# Autodesk Inventor assembly: ヘラ
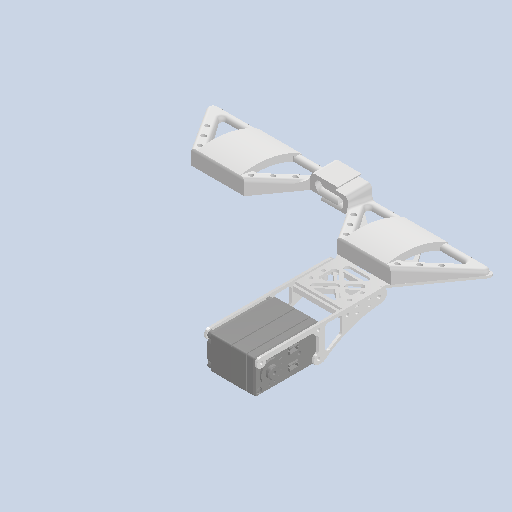
[picture p0: Inventor's stored thumbnail of the model, 512x512]
Saved by Autodesk Inventor 2024 (Build 280153000, 153)
## iProperties
Created: 2023-08-01
Part Number: ヘラ
Document SubType Name: Assembly
Designer: right
Mass: 56.6526 g
Surface Area: 176.367 cm^2
Volume: 31.3921 cm^3
Density: 1.80467 g/cm^3
Author: right
## Documents named in this file (7)
- C:\Users\right\OneDrive\ドキュメント\Inventor\V2二足Light＿仮\ヘラ.iam
- C:\Users\right\OneDrive\ドキュメント\Inventor\V2二足Light＿仮\KRS2500_scale.ipt
- C:\Users\right\OneDrive\ドキュメント\Inventor\V2二足Light＿仮\hera_nemoto.ipt
- C:\Users\right\OneDrive\ドキュメント\Inventor\V2二足Light＿仮\heraosae.ipt
- C:\Users\right\OneDrive\ドキュメント\Inventor\V2二足Light＿仮\hera.ipt
- C:\Users\right\OneDrive\ドキュメント\Inventor\V2二足Light＿仮\heraue_2.ipt
- C:\Users\right\OneDrive\ドキュメント\Inventor\V2二足Light＿仮\heraue_2_MIR.ipt
## Components (7 placed, 6 different names)
1. KRS2500_scale:1 — メイト:1, メイト:2, フラッシュ:1, フラッシュ:2, 挿入:3, 挿入:4, 挿入:5, 挿入:6
2. hera_nemoto:1 — フラッシュ:2, 挿入:3, 挿入:4, 挿入:7, 挿入:8
3. hera_nemoto:2 — 挿入:5, 挿入:6, 挿入:9, 挿入:10
4. heraosae:1 — 挿入:7, 挿入:8, 挿入:9, 挿入:10, フラッシュ:3
5. hera:1 — フラッシュ:3, フラッシュ:4
6. heraue_2:1 — フラッシュ:4, メイト:3, 角度:1, フラッシュ:5
7. heraue_2_MIR:1 — メイト:3, 角度:1, フラッシュ:5
## Relationships (17: Insert 8, Flush 5, Mate 3, Angle 1)
- メイト:1 [Mate]: KRS2500_scale:1
- メイト:2 [Mate]: KRS2500_scale:1
- フラッシュ:1 [Flush]: KRS2500_scale:1
- フラッシュ:2 [Flush]: KRS2500_scale:1 ↔ hera_nemoto:1
- 挿入:3 [Insert]: KRS2500_scale:1 ↔ hera_nemoto:1
- 挿入:4 [Insert]: KRS2500_scale:1 ↔ hera_nemoto:1
- 挿入:5 [Insert]: KRS2500_scale:1 ↔ hera_nemoto:2
- 挿入:6 [Insert]: KRS2500_scale:1 ↔ hera_nemoto:2
- 挿入:7 [Insert]: hera_nemoto:1 ↔ heraosae:1
- 挿入:8 [Insert]: hera_nemoto:1 ↔ heraosae:1
- 挿入:9 [Insert]: hera_nemoto:2 ↔ heraosae:1
- 挿入:10 [Insert]: hera_nemoto:2 ↔ heraosae:1
- フラッシュ:3 [Flush]: heraosae:1 ↔ hera:1
- フラッシュ:4 [Flush]: hera:1 ↔ heraue_2:1
- メイト:3 [Mate]: heraue_2:1 ↔ heraue_2_MIR:1
- 角度:1 [Angle] (0 deg): heraue_2:1 ↔ heraue_2_MIR:1
- フラッシュ:5 [Flush]: heraue_2:1 ↔ heraue_2_MIR:1
